# Autodesk Inventor assembly: Сборка4
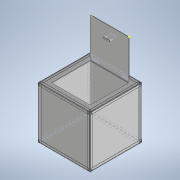
[picture p0: Inventor's stored thumbnail of the model, 180x180]
Saved by Autodesk Inventor 2022 (Build 260153000, 153)
## iProperties
Created: 2023-02-17
Part Number: Сборка4
Document SubType Name: Assembly
Designer: 89684288964
Author: 89684288964
## Documents named in this file (6)
- C:\Users\89684288964\Desktop\Сборка4.iam
- C:\Users\89684288964\Desktop\8.ipt
- C:\Users\89684288964\Desktop\9.ipt
- C:\Users\89684288964\Desktop\0.ipt
- C:\Users\89684288964\Desktop\5.ipt
- C:\Users\89684288964\Desktop\2.ipt
## Components (19 placed, 5 different names)
1. 8:1 — Совмещение:1, Заподлицо:1, Совмещение:2, Совмещение:6, Совмещение:7, Совмещение:8, Совмещение:15, Совмещение:16, Заподлицо:9, Совмещение:35, Совмещение:37
2. 9:1 — Совмещение:1, Заподлицо:1, Совмещение:2, Совмещение:3, Совмещение:4, Заподлицо:2, Совмещение:27, Совмещение:36, Совмещение:41
3. 8:2 — Совмещение:3, Совмещение:4, Совмещение:5, Заподлицо:8, Совмещение:30
4. 9:2 — Совмещение:5, Совмещение:6, Заподлицо:9, Заподлицо:10, Совмещение:34, Совмещение:45
5. 9:3 — Совмещение:7, Совмещение:8, Заподлицо:2, Совмещение:43
6. 9:6 — Совмещение:15, Совмещение:16, Совмещение:39, Совмещение:46
7. 8:5 — Заподлицо:6, Заподлицо:7
8. 9:10 — Совмещение:32, Совмещение:42
9. 8:6 — Совмещение:33, Совмещение:38
10. 9:11 — Заподлицо:6, Совмещение:31, Совмещение:44
11. 9:12 — Заподлицо:8
12. 9:13 — Заподлицо:7, Совмещение:27, Заподлицо:10, Совмещение:28, Совмещение:29
13. 0:1 — Совмещение:28, Совмещение:29, Совмещение:30
14. 0:2 — Совмещение:31, Совмещение:32, Совмещение:33
15. 0:3 — Совмещение:34, Совмещение:35, Совмещение:36
16. 5:1 — Совмещение:37, Совмещение:38, Совмещение:39, Совмещение:40
17. 2:1 — Совмещение:40
18. 0:4 — Совмещение:41, Совмещение:42, Совмещение:43
19. 0:5 — Совмещение:44, Совмещение:45, Совмещение:46
## Relationships (49: Mate 40, Flush 9)
- Совмещение:1 [Mate]: 8:1 ↔ 9:1
- Заподлицо:1 [Flush]: 8:1 ↔ 9:1
- Совмещение:2 [Mate]: 8:1 ↔ 9:1
- Совмещение:3 [Mate]: 9:1 ↔ 8:2
- Совмещение:4 [Mate]: 9:1 ↔ 8:2
- Совмещение:5 [Mate]: 8:2 ↔ 9:2
- Совмещение:6 [Mate]: 8:1 ↔ 9:2
- Совмещение:7 [Mate]: 8:1 ↔ 9:3
- Совмещение:8 [Mate]: 8:1 ↔ 9:3
- Заподлицо:2 [Flush]: 9:1 ↔ 9:3
- Совмещение:15 [Mate]: 8:1 ↔ 9:6
- Совмещение:16 [Mate]: 8:1 ↔ 9:6
- [Mate]: 8:5 ↔ 9:10
- [Flush]: 8:5 ↔ 9:10
- [Mate]: 8:5 ↔ 9:10
- [Mate]: 9:10 ↔ 8:6
- [Mate]: 9:10 ↔ 8:6
- [Mate]: 8:6 ↔ 9:11
- [Mate]: 8:5 ↔ 9:11
- [Mate]: 8:5 ↔ 9:12
- [Mate]: 8:5 ↔ 9:12
- [Flush]: 9:10 ↔ 9:12
- [Mate]: 8:5 ↔ 9:13
- [Mate]: 8:5 ↔ 9:13
- Заподлицо:6 [Flush]: 8:5 ↔ 9:11
- Заподлицо:7 [Flush]: 8:5 ↔ 9:13
- Совмещение:27 [Mate]: 9:1 ↔ 9:13
- Заподлицо:8 [Flush]: 8:2 ↔ 9:12
- Заподлицо:9 [Flush]: 8:1 ↔ 9:2
- Заподлицо:10 [Flush]: 9:2 ↔ 9:13
- Совмещение:28 [Mate]: 9:13 ↔ 0:1
- Совмещение:29 [Mate]: 9:13 ↔ 0:1
- Совмещение:30 [Mate]: 8:2 ↔ 0:1
- Совмещение:31 [Mate]: 9:11 ↔ 0:2
- Совмещение:32 [Mate]: 9:10 ↔ 0:2
- Совмещение:33 [Mate]: 8:6 ↔ 0:2
- Совмещение:34 [Mate]: 9:2 ↔ 0:3
- Совмещение:35 [Mate]: 8:1 ↔ 0:3
- Совмещение:36 [Mate]: 9:1 ↔ 0:3
- Совмещение:37 [Mate]: 8:1 ↔ 5:1
- Совмещение:38 [Mate]: 8:6 ↔ 5:1
- Совмещение:39 [Mate]: 9:6 ↔ 5:1
- Совмещение:40 [Mate]: 5:1 ↔ 2:1
- Совмещение:41 [Mate]: 9:1 ↔ 0:4
- Совмещение:42 [Mate]: 9:10 ↔ 0:4
- Совмещение:43 [Mate]: 9:3 ↔ 0:4
- Совмещение:44 [Mate]: 9:11 ↔ 0:5
- Совмещение:45 [Mate]: 9:2 ↔ 0:5
- Совмещение:46 [Mate]: 9:6 ↔ 0:5
## Named parameters: d29_d13 = 0 mm, d30_d14 = 0 mm, d31_d15 = 0 mm, d32_d16 = 0 mm, d33_d17 = 0 mm, d34_d18 = 0 mm, d35_d19 = 0 mm, d36_d27 = 0 mm, d37_d28 = 0 mm, d38_d10 = 0 mm, d39_d11 = 0 mm, d40_d12 = 0 mm
